# Autodesk Inventor assembly: herramienta_final
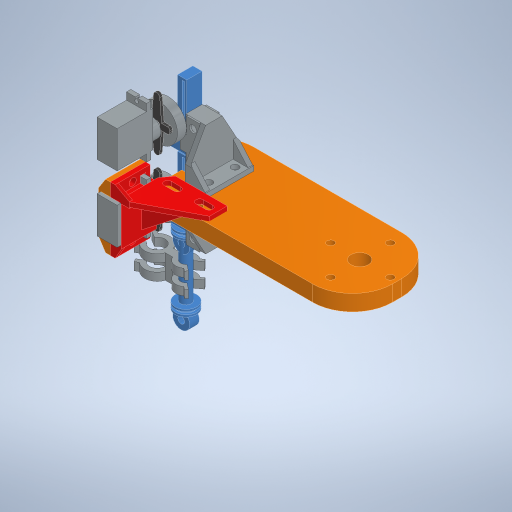
[picture p0: Inventor's stored thumbnail of the model, 512x512]
Saved by Autodesk Inventor 2024.3 (Build 283343000, 343)
## iProperties
Created: 2024-10-01
Part Number: herramienta_final
Document SubType Name: Assembly
Designer: User
Author: User
## Documents named in this file (5)
- C:\Users\User\Documents\Universidad Octavo Semestre\Robotica Industrial\matlab\SCARA\mariana_scara_final\mariana_scara_final\herramienta_final.iam
- C:\Users\User\Documents\Universidad Octavo Semestre\Robotica Industrial\matlab\SCARA\mariana_scara_final\mariana_scara_final\pinza.iam
- C:\Users\User\Documents\Universidad Octavo Semestre\Robotica Industrial\matlab\SCARA\mariana_scara_final\mariana_scara_final\soporte-motor.ipt
- C:\Users\User\Documents\Universidad Octavo Semestre\Robotica Industrial\matlab\SCARA\mariana_scara_final\mariana_scara_final\soprte_motor.ipt
- C:\Users\User\Documents\Universidad Octavo Semestre\Robotica Industrial\matlab\SCARA\mariana_scara_final\mariana_scara_final\lamina_herrAMIENTA.ipt
## Components (4 placed, 4 different names)
1. pinza:1 [sub-assembly] — Mate:2, Mate:3, Flush:3, Mate:4, Mate:5, Mate:6
2. soporte-motor:1 — Mate:1, Flush:1, Flush:2, Mate:3, Flush:3
3. soprte_motor:1 — Mate:1, Flush:1, Flush:2, Mate:2
4. lamina_herrAMIENTA:1 — Mate:4, Mate:5, Mate:6
## Relationships (9: Mate 6, Flush 3)
- Mate:1: soporte-motor:1 ↔ soprte_motor:1
- Flush:1: soporte-motor:1 ↔ soprte_motor:1
- Flush:2: soporte-motor:1 ↔ soprte_motor:1
- Mate:2: pinza:1 ↔ soprte_motor:1
- Mate:3: pinza:1 ↔ soporte-motor:1
- Flush:3 (2.34 mm): pinza:1 ↔ soporte-motor:1
- Mate:4 (-8 mm): pinza:1 ↔ lamina_herrAMIENTA:1
- Mate:5: pinza:1 ↔ lamina_herrAMIENTA:1
- Mate:6: pinza:1 ↔ lamina_herrAMIENTA:1
